# Autodesk Inventor assembly: Sensor Mount Film Applicator - V1
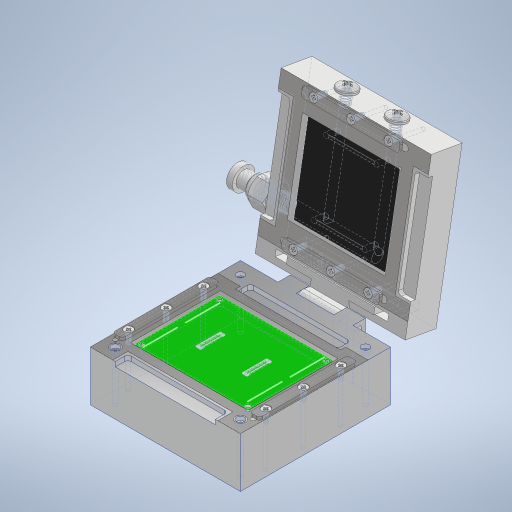
[picture p0: Inventor's stored thumbnail of the model, 512x512]
Saved by Autodesk Inventor 2023 (Build 270158000, 158)
## iProperties
Created: 2022-06-13
Part Number: Sensor Mount Film Applicator - V1
Document SubType Name: Assembly
Designer: Caleb
Author: Caleb
## Documents named in this file (13)
- C:\Users\Caleb\Desktop\nebraska-silicon-lab\Hardware\ETL\Jigs\Sensor Mount Film Applicator\Sensor Mount Film Applicator - V1.iam
- C:\Users\Caleb\Desktop\nebraska-silicon-lab\Hardware\ETL\Jigs\Sensor Mount Film Applicator\Base - V1.ipt
- C:\Users\Caleb\Desktop\nebraska-silicon-lab\Hardware\ETL\Jigs\Sensor Mount Film Applicator\Hinge - V1.ipt
- C:\Users\Caleb\Desktop\nebraska-silicon-lab\Hardware\ETL\Jigs\Sensor Mount Film Applicator\Top - V1.ipt
- C:\Users\Caleb\Desktop\nebraska-silicon-lab\Hardware\ETL\Jigs\Sensor Mount Film Applicator\Pin - V1.ipt
- C:\Users\Caleb\Desktop\nebraska-silicon-lab\Hardware\ETL\modules\tamale v1.3\Mock Module PCB - v1p3.iam
- C:\Users\Caleb\Desktop\nebraska-silicon-lab\Hardware\ETL\modules\tamale v1.3\Sensor Placement Film.ipt
- C:\Users\Caleb\Desktop\nebraska-silicon-lab\Hardware\ETL\Jigs\Sensor Mount Film Applicator\Module PCB Stencil - V1.ipt
- C:\Users\Caleb\Desktop\nebraska-silicon-lab\Hardware\ETL\Jigs\Sensor Mount Film Applicator\Stencil Clamp - V1.ipt
- C:\Users\Caleb\Desktop\nebraska-silicon-lab\Hardware\ETL\Jigs\Sensor Mount Film Applicator\91099A104_Passivated 18-8 Stainless Steel Phillips Flat Head Screw.ipt
- C:\Users\Caleb\Desktop\nebraska-silicon-lab\Hardware\ETL\Jigs\Sensor Mount Film Applicator\Sensor Mount Film Stencil - V1.ipt
- C:\Users\Caleb\Desktop\nebraska-silicon-lab\Hardware\ETL\Jigs\Sensor Mount Film Applicator\51025K323_Brass Push-to-Connect Tube Fitting for Air.ipt
- C:\Users\Caleb\Desktop\nebraska-silicon-lab\Hardware\ETL\Jigs\Sensor Mount Film Applicator\91772A238_Passivated 18-8 Stainless Steel Pan Head Phillips Screw.ipt
## Components (27 placed, 12 different names)
1. Base - V1:1 — Insert:1, Mate:3, Mate:8, Flush:2, Flush:3
2. Hinge - V1:1 — Rigid:1, Mate:1, Mate:2, Flush:1
3. Top - V1:1 — Mate:1, Mate:2, Flush:1, Mate:5, Mate:11, Flush:4, Flush:5, Angle:1, Angle:2, Flush:6, Flush:7, Flush:8, Flush:9, Insert:14, Insert:15, Insert:16
4. Pin - V1:1 — Insert:1, Rigid:1
5. Mock Module PCB - v1p3:1 [sub-assembly] — Mate:3, Mate:14, Mate:15
6. Sensor Placement Film:1 — Mate:5, Mate:16, Mate:17
7. Module PCB Stencil - V1:1 — Mate:8, Flush:2, Flush:3, Mate:9, Mate:10, Mate:14, Mate:15, Angle:3
8. Stencil Clamp - V1:1 — Mate:9, Insert:2, Insert:3, Insert:4
9. 91099A104_Passivated 18-8 Stainless Steel Phillips Flat Head Screw:1 — Insert:2
10. 91099A104_Passivated 18-8 Stainless Steel Phillips Flat Head Screw:2 — Insert:3
11. 91099A104_Passivated 18-8 Stainless Steel Phillips Flat Head Screw:3 — Insert:4
12. Stencil Clamp - V1:2 — Mate:10, Insert:5, Insert:6, Insert:7
13. 91099A104_Passivated 18-8 Stainless Steel Phillips Flat Head Screw:4 — Insert:5
14. 91099A104_Passivated 18-8 Stainless Steel Phillips Flat Head Screw:5 — Insert:6
15. 91099A104_Passivated 18-8 Stainless Steel Phillips Flat Head Screw:6 — Insert:7
16. Sensor Mount Film Stencil - V1:1 — Mate:11, Flush:4, Flush:5, Mate:12, Mate:13, Mate:16, Mate:17, Angle:3
17. Stencil Clamp - V1:3 — Mate:13, Angle:2, Flush:6, Flush:7, Insert:11, Insert:12, Insert:13
18. Stencil Clamp - V1:4 — Mate:12, Angle:1, Flush:8, Flush:9, Insert:8, Insert:9, Insert:10
19. 91099A104_Passivated 18-8 Stainless Steel Phillips Flat Head Screw:7 — Insert:10
20. 91099A104_Passivated 18-8 Stainless Steel Phillips Flat Head Screw:8 — Insert:8
21. 91099A104_Passivated 18-8 Stainless Steel Phillips Flat Head Screw:9 — Insert:9
22. 91099A104_Passivated 18-8 Stainless Steel Phillips Flat Head Screw:10 — Insert:11
23. 91099A104_Passivated 18-8 Stainless Steel Phillips Flat Head Screw:11 — Insert:12
24. 91099A104_Passivated 18-8 Stainless Steel Phillips Flat Head Screw:12 — Insert:13
25. 51025K323_Brass Push-to-Connect Tube Fitting for Air:1 — Insert:14
26. 91772A238_Passivated 18-8 Stainless Steel Pan Head Phillips Screw:1 — Insert:15
27. 91772A238_Passivated 18-8 Stainless Steel Pan Head Phillips Screw:2 — Insert:16
## Relationships (43: Insert 16, Mate 14, Flush 9, Angle 3, WeldJoint 1)
- Insert:1: Base - V1:1 ↔ Pin - V1:1
- Rigid:1 [WeldJoint] (9.525 mm): Hinge - V1:1 ↔ Pin - V1:1
- Mate:1: Hinge - V1:1 ↔ Top - V1:1
- Mate:2: Hinge - V1:1 ↔ Top - V1:1
- Flush:1 (3.81 mm): Hinge - V1:1 ↔ Top - V1:1
- Mate:3: Base - V1:1 ↔ Mock Module PCB - v1p3:1
- Mate:5: Top - V1:1 ↔ Sensor Placement Film:1
- Mate:8: Base - V1:1 ↔ Module PCB Stencil - V1:1
- Flush:2: Base - V1:1 ↔ Module PCB Stencil - V1:1
- Flush:3: Base - V1:1 ↔ Module PCB Stencil - V1:1
- Mate:9: Module PCB Stencil - V1:1 ↔ Stencil Clamp - V1:1
- Insert:2: Stencil Clamp - V1:1 ↔ 91099A104_Passivated 18-8 Stainless Steel Phillips Flat Head Screw:1
- Insert:3: Stencil Clamp - V1:1 ↔ 91099A104_Passivated 18-8 Stainless Steel Phillips Flat Head Screw:2
- Insert:4: Stencil Clamp - V1:1 ↔ 91099A104_Passivated 18-8 Stainless Steel Phillips Flat Head Screw:3
- Mate:10: Module PCB Stencil - V1:1 ↔ Stencil Clamp - V1:2
- Insert:5: Stencil Clamp - V1:2 ↔ 91099A104_Passivated 18-8 Stainless Steel Phillips Flat Head Screw:4
- Insert:6: Stencil Clamp - V1:2 ↔ 91099A104_Passivated 18-8 Stainless Steel Phillips Flat Head Screw:5
- Insert:7: Stencil Clamp - V1:2 ↔ 91099A104_Passivated 18-8 Stainless Steel Phillips Flat Head Screw:6
- Mate:11: Top - V1:1 ↔ Sensor Mount Film Stencil - V1:1
- Flush:4: Top - V1:1 ↔ Sensor Mount Film Stencil - V1:1
- Flush:5: Top - V1:1 ↔ Sensor Mount Film Stencil - V1:1
- Mate:12: Sensor Mount Film Stencil - V1:1 ↔ Stencil Clamp - V1:4
- Mate:13: Sensor Mount Film Stencil - V1:1 ↔ Stencil Clamp - V1:3
- Angle:1 (0 deg): Top - V1:1 ↔ Stencil Clamp - V1:4
- Angle:2 (0 deg): Top - V1:1 ↔ Stencil Clamp - V1:3
- Flush:6 (0.635 mm): Top - V1:1 ↔ Stencil Clamp - V1:3
- Flush:7 (13.97 mm): Top - V1:1 ↔ Stencil Clamp - V1:3
- Flush:8 (8.255 mm): Top - V1:1 ↔ Stencil Clamp - V1:4
- Flush:9 (13.462 mm): Top - V1:1 ↔ Stencil Clamp - V1:4
- Insert:8: Stencil Clamp - V1:4 ↔ 91099A104_Passivated 18-8 Stainless Steel Phillips Flat Head Screw:8
- Insert:9: Stencil Clamp - V1:4 ↔ 91099A104_Passivated 18-8 Stainless Steel Phillips Flat Head Screw:9
- Insert:10: Stencil Clamp - V1:4 ↔ 91099A104_Passivated 18-8 Stainless Steel Phillips Flat Head Screw:7
- Insert:11: Stencil Clamp - V1:3 ↔ 91099A104_Passivated 18-8 Stainless Steel Phillips Flat Head Screw:10
- Insert:12: Stencil Clamp - V1:3 ↔ 91099A104_Passivated 18-8 Stainless Steel Phillips Flat Head Screw:11
- Insert:13: Stencil Clamp - V1:3 ↔ 91099A104_Passivated 18-8 Stainless Steel Phillips Flat Head Screw:12
- Mate:14: Mock Module PCB - v1p3:1 ↔ Module PCB Stencil - V1:1
- Mate:15: Mock Module PCB - v1p3:1 ↔ Module PCB Stencil - V1:1
- Mate:16: Sensor Placement Film:1 ↔ Sensor Mount Film Stencil - V1:1
- Mate:17: Sensor Placement Film:1 ↔ Sensor Mount Film Stencil - V1:1
- Insert:14: Top - V1:1 ↔ 51025K323_Brass Push-to-Connect Tube Fitting for Air:1
- Insert:15: Top - V1:1 ↔ 91772A238_Passivated 18-8 Stainless Steel Pan Head Phillips Screw:1
- Insert:16: Top - V1:1 ↔ 91772A238_Passivated 18-8 Stainless Steel Pan Head Phillips Screw:2
- Angle:3 (-80 deg): Module PCB Stencil - V1:1 ↔ Sensor Mount Film Stencil - V1:1
